# Autodesk Inventor assembly: accembly
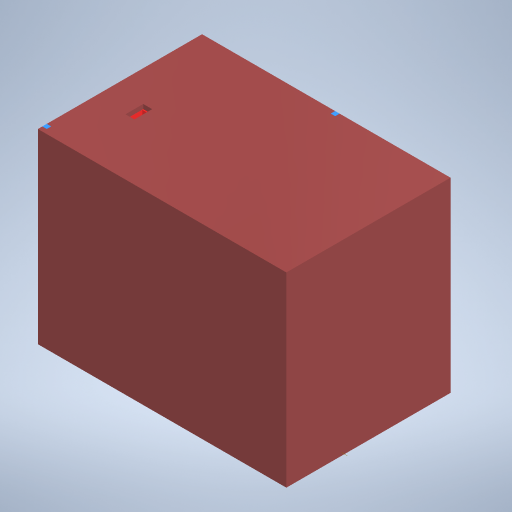
[picture p0: Inventor's stored thumbnail of the model, 512x512]
Saved by Autodesk Inventor 2024 (Build 280153000, 153)
## iProperties
Created: 2024-04-17
Part Number: accembly
Document SubType Name: Assembly
Designer: 22546723
Author: 22546723
## Documents named in this file (6)
- H:\skripsie\inventor\accembly.iam
- H:\skripsie\inventor\case.ipt
- H:\skripsie\inventor\lid.ipt
- H:\skripsie\inventor\pump.ipt
- H:\skripsie\inventor\battery_pack.ipt
- H:\skripsie\inventor\esp.ipt
## Components (5 placed, 5 different names)
1. case:1 — Mate:1, Flush:1, Mate:2, Mate:3, Flush:2, Mate:4, Mate:5, Mate:6
2. lid:1 — Mate:1, Flush:1
3. pump:1 — Mate:4, Mate:5
4. battery_pack:1 — Mate:2, Mate:3, Flush:2
5. esp:1 — Mate:6
## Relationships (8: Mate 6, Flush 2)
- Mate:1: case:1 ↔ lid:1
- Flush:1: case:1 ↔ lid:1
- Mate:2: case:1 ↔ battery_pack:1
- Mate:3 (1 mm): case:1 ↔ battery_pack:1
- Flush:2: case:1 ↔ battery_pack:1
- Mate:4: case:1 ↔ pump:1
- Mate:5: case:1 ↔ pump:1
- Mate:6: case:1 ↔ esp:1
